# Autodesk Inventor assembly: macropad
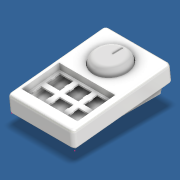
[picture p0: Inventor's stored thumbnail of the model, 180x180]
Saved by Autodesk Inventor 2020 (Build 240168000, 168)
## iProperties
Created: 2021-08-07
Part Number: macropad
Document SubType Name: Assembly
Designer: RNG3nius
Author: RNG3nius
## Documents named in this file (4)
- G:\Projects\Macropad\macropad.iam
- G:\Projects\Macropad\Top shell.ipt
- G:\Projects\Macropad\Bottom.ipt
- G:\Projects\Macropad\knob.ipt
## Components (3 placed, 3 different names)
1. Bottom:1 — Mate:1, Mate:6, Mate:7, Mate:8, Mate:9
2. knob:1 — Mate:10, Mate:11, Mate:12
3. Top shell:1 — Mate:7, Mate:8, Mate:9, Mate:10, Mate:11, Mate:12
## Relationships (8: Mate 8)
- Mate:1: Bottom:1
- Mate:6: Bottom:1
- Mate:7: Bottom:1 ↔ Top shell:1
- Mate:8: Bottom:1 ↔ Top shell:1
- Mate:9: Bottom:1 ↔ Top shell:1
- Mate:10: knob:1 ↔ Top shell:1
- Mate:11: knob:1 ↔ Top shell:1
- Mate:12: knob:1 ↔ Top shell:1
